# Autodesk Inventor assembly: ArcadeController
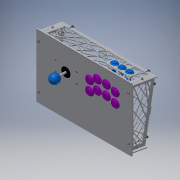
[picture p0: Inventor's stored thumbnail of the model, 180x180]
Saved by Autodesk Inventor 2019 (Build 230136000, 136)
## iProperties
Created: 2013-02-02
Part Number: ArcadeController
Document SubType Name: Assembly
Designer: xylzlyx
Author: xylzlyx
## Documents named in this file (14)
- D:\GitRepos\Pew-Pew-Stick\inventor\assemblies\ArcadeController.iam
- D:\GitRepos\Pew-Pew-Stick\inventor\parts\Panel_top.ipt
- D:\GitRepos\Pew-Pew-Stick\inventor\parts\Panel_bottom.ipt
- D:\GitRepos\Pew-Pew-Stick\inventor\parts\JLF-TP-8YT_body.ipt
- D:\GitRepos\Pew-Pew-Stick\inventor\parts\JLF-TP-8YT_ball.ipt
- D:\GitRepos\Pew-Pew-Stick\inventor\parts\JLF-TP-8YT_ring.ipt
- D:\GitRepos\Pew-Pew-Stick\inventor\parts\OBSF-30-B_button.ipt
- D:\GitRepos\Pew-Pew-Stick\inventor\parts\Panel_back.ipt
- D:\GitRepos\Pew-Pew-Stick\inventor\parts\Panel_front.ipt
- D:\GitRepos\Pew-Pew-Stick\inventor\parts\Panel_side.ipt
- D:\GitRepos\Pew-Pew-Stick\inventor\parts\OBSF-24_button.ipt
- C:\Users\mstine\Documents\Inventor\Content Center Files\R2019\en-US\ANSI B18.22.1\ANSI B18.22.1 - No. 6 - Type A.ipt
- C:\Users\mstine\Documents\Inventor\Content Center Files\R2019\en-US\ANSI B18.3(05)\ANSI B18.3 - 6-32 UNC - 0.5(31).ipt
- D:\GitRepos\Pew-Pew-Stick\inventor\assemblies\ArcadeController\Design Accelerator\Bolted Connection2.iam
## Components (53 placed, 13 different names)
1. TopPanel:1 — Flush:1, Flush:2, Insert:1, Insert:2, Insert:4, Insert:5, Insert:6, Insert:7, Insert:8, Insert:9, Insert:10, Insert:11, Insert:12, Mate:6, Mate:10, Insert:14, Insert:17, Insert:18, Insert:19, Mate:14, Mate:15
2. BottomPanel:1 — Flush:1, Flush:2, Mate:3, Flush:3, Flush:4, Flush:5, Flush:6, Flush:8, Flush:9, Mate:4, Mate:5, Flush:10, Flush:12, Flush:13, Mate:8, Flush:14, Mate:13, Insert:22, Insert:23, Insert:24, Insert:25, Insert:26, Insert:27, Insert:28, Insert:29
3. JLF-TP-8YT_body:1 — Insert:1, Insert:2, Insert:3, Mate:3
4. JoystickBall:1 — Insert:3
5. JoystickCover:1 — Insert:4
6. OBSF-30-B_button:1 — Insert:5
7. OBSF-30-B_button:2 — Insert:6
8. OBSF-30-B_button:3 — Insert:7
9. OBSF-30-B_button:4 — Insert:8
10. OBSF-30-B_button:5 — Insert:9
11. OBSF-30-B_button:6 — Insert:10
12. OBSF-30-B_button:7 — Insert:11
13. OBSF-30-B_button:8 — Insert:12
14. Panel_back:1 — Flush:3, Flush:4, Mate:5, Flush:10, Mate:11, Mate:12, Insert:15, Insert:16, Insert:45, Insert:46, Insert:47
15. Panel_front:1 — Flush:5, Flush:6, Flush:12, Mate:9, Flush:14, Mate:13, Insert:20, Insert:21
16. Panel_side:1 — Flush:8, Flush:9, Mate:4, Mate:6, Mate:12
17. Panel_side:2 — Flush:13, Mate:8, Mate:9, Mate:10, Mate:11
18. Hexagon Socket Head Cap Screw - Inch No. 6 - 32 UNC - 1/2:20 — Insert:13
19. Plain Washer (Inch) No. 6 - Type A:17 — Insert:13, Insert:14
20. Hexagon Socket Head Cap Screw - Inch No. 6 - 32 UNC - 1/2:21 — Insert:30
21. Plain Washer (Inch) No. 6 - Type A:18 — Insert:15, Insert:31
22. Hexagon Socket Head Cap Screw - Inch No. 6 - 32 UNC - 1/2:22 — Insert:31
23. Plain Washer (Inch) No. 6 - Type A:19 — Insert:16, Insert:30
24. Hexagon Socket Head Cap Screw - Inch No. 6 - 32 UNC - 1/2:23 — Insert:32
25. Plain Washer (Inch) No. 6 - Type A:20 — Insert:17, Insert:35
26. Hexagon Socket Head Cap Screw - Inch No. 6 - 32 UNC - 1/2:24 — Insert:33
27. Plain Washer (Inch) No. 6 - Type A:21 — Insert:19, Insert:32
28. Hexagon Socket Head Cap Screw - Inch No. 6 - 32 UNC - 1/2:25 — Insert:34
29. Plain Washer (Inch) No. 6 - Type A:22 — Insert:18, Insert:34
30. Plain Washer (Inch) No. 6 - Type A:23 — Insert:20, Insert:33
31. Plain Washer (Inch) No. 6 - Type A:24 — Insert:21, Insert:36
32. Plain Washer (Inch) No. 6 - Type A:25 — Insert:25, Insert:43
33. Plain Washer (Inch) No. 6 - Type A:26 — Insert:24, Insert:44
34. Plain Washer (Inch) No. 6 - Type A:27 — Insert:23, Insert:39
35. Plain Washer (Inch) No. 6 - Type A:28 — Insert:22, Insert:40
36. Plain Washer (Inch) No. 6 - Type A:29 — Insert:26, Insert:37
37. Plain Washer (Inch) No. 6 - Type A:30 — Insert:27, Insert:38
38. Plain Washer (Inch) No. 6 - Type A:31 — Insert:28, Insert:41
39. Plain Washer (Inch) No. 6 - Type A:32 — Insert:29, Insert:42
40. Hexagon Socket Head Cap Screw - Inch No. 6 - 32 UNC - 1/2:26 — Insert:40
41. Hexagon Socket Head Cap Screw - Inch No. 6 - 32 UNC - 1/2:27 — Insert:35
42. Hexagon Socket Head Cap Screw - Inch No. 6 - 32 UNC - 1/2:28 — Insert:36
43. Hexagon Socket Head Cap Screw - Inch No. 6 - 32 UNC - 1/2:29 — Insert:37
44. Hexagon Socket Head Cap Screw - Inch No. 6 - 32 UNC - 1/2:30 — Insert:39
45. Hexagon Socket Head Cap Screw - Inch No. 6 - 32 UNC - 1/2:31 — Insert:38
46. Hexagon Socket Head Cap Screw - Inch No. 6 - 32 UNC - 1/2:32 — Insert:42
47. Hexagon Socket Head Cap Screw - Inch No. 6 - 32 UNC - 1/2:33 — Insert:41
48. Hexagon Socket Head Cap Screw - Inch No. 6 - 32 UNC - 1/2:34 — Insert:43
49. Hexagon Socket Head Cap Screw - Inch No. 6 - 32 UNC - 1/2:35 — Insert:44
50. OBSF-24_button:1 — Insert:45
51. OBSF-24_button:2 — Insert:46
52. OBSF-24_button:3 — Insert:47
53. Bolted Connection:1 [sub-assembly] — Mate:14, Mate:15
## Relationships (71: Insert 47, Flush 12, Mate 12)
- Flush:1: TopPanel:1 ↔ BottomPanel:1
- Flush:2: TopPanel:1 ↔ BottomPanel:1
- Insert:1: TopPanel:1 ↔ JLF-TP-8YT_body:1
- Insert:2: TopPanel:1 ↔ JLF-TP-8YT_body:1
- Insert:3: JLF-TP-8YT_body:1 ↔ JoystickBall:1
- Insert:4: TopPanel:1 ↔ JoystickCover:1
- Insert:5: TopPanel:1 ↔ OBSF-30-B_button:1
- Insert:6: TopPanel:1 ↔ OBSF-30-B_button:2
- Insert:7: TopPanel:1 ↔ OBSF-30-B_button:3
- Insert:8: TopPanel:1 ↔ OBSF-30-B_button:4
- Insert:9: TopPanel:1 ↔ OBSF-30-B_button:5
- Insert:10: TopPanel:1 ↔ OBSF-30-B_button:6
- Insert:11: TopPanel:1 ↔ OBSF-30-B_button:7
- Insert:12: TopPanel:1 ↔ OBSF-30-B_button:8
- Mate:3 (44.45 mm): BottomPanel:1 ↔ JLF-TP-8YT_body:1
- Flush:3: BottomPanel:1 ↔ Panel_back:1
- Flush:4 (-12.7 mm): BottomPanel:1 ↔ Panel_back:1
- Flush:5: BottomPanel:1 ↔ Panel_front:1
- Flush:6 (-9.525 mm): BottomPanel:1 ↔ Panel_front:1
- Flush:8 (-9.525 mm): BottomPanel:1 ↔ Panel_side:1
- Flush:9 (9.525 mm): BottomPanel:1 ↔ Panel_side:1
- Mate:4: BottomPanel:1 ↔ Panel_side:1
- Mate:5: BottomPanel:1 ↔ Panel_back:1
- Flush:10: BottomPanel:1 ↔ Panel_back:1
- Mate:6: TopPanel:1 ↔ Panel_side:1
- Flush:12 (9.525 mm): BottomPanel:1 ↔ Panel_front:1
- Flush:13 (9.525 mm): BottomPanel:1 ↔ Panel_side:2
- Mate:8: BottomPanel:1 ↔ Panel_side:2
- Mate:9: Panel_front:1 ↔ Panel_side:2
- Mate:10: TopPanel:1 ↔ Panel_side:2
- Mate:11: Panel_back:1 ↔ Panel_side:2
- Mate:12: Panel_back:1 ↔ Panel_side:1
- Flush:14: BottomPanel:1 ↔ Panel_front:1
- Mate:13: BottomPanel:1 ↔ Panel_front:1
- Insert:13: Hexagon Socket Head Cap Screw - Inch No. 6 - 32 UNC - 1/2:20 ↔ Plain Washer (Inch) No. 6 - Type A:17
- Insert:14: TopPanel:1 ↔ Plain Washer (Inch) No. 6 - Type A:17
- Insert:15: Panel_back:1 ↔ Plain Washer (Inch) No. 6 - Type A:18
- Insert:16: Panel_back:1 ↔ Plain Washer (Inch) No. 6 - Type A:19
- Insert:17: TopPanel:1 ↔ Plain Washer (Inch) No. 6 - Type A:20
- Insert:18: TopPanel:1 ↔ Plain Washer (Inch) No. 6 - Type A:22
- Insert:19: TopPanel:1 ↔ Plain Washer (Inch) No. 6 - Type A:21
- Insert:20: Panel_front:1 ↔ Plain Washer (Inch) No. 6 - Type A:23
- Insert:21: Panel_front:1 ↔ Plain Washer (Inch) No. 6 - Type A:24
- Insert:22: BottomPanel:1 ↔ Plain Washer (Inch) No. 6 - Type A:28
- Insert:23: BottomPanel:1 ↔ Plain Washer (Inch) No. 6 - Type A:27
- Insert:24: BottomPanel:1 ↔ Plain Washer (Inch) No. 6 - Type A:26
- Insert:25: BottomPanel:1 ↔ Plain Washer (Inch) No. 6 - Type A:25
- Insert:26: BottomPanel:1 ↔ Plain Washer (Inch) No. 6 - Type A:29
- Insert:27: BottomPanel:1 ↔ Plain Washer (Inch) No. 6 - Type A:30
- Insert:28: BottomPanel:1 ↔ Plain Washer (Inch) No. 6 - Type A:31
- Insert:29: BottomPanel:1 ↔ Plain Washer (Inch) No. 6 - Type A:32
- Insert:30: Hexagon Socket Head Cap Screw - Inch No. 6 - 32 UNC - 1/2:21 ↔ Plain Washer (Inch) No. 6 - Type A:19
- Insert:31: Plain Washer (Inch) No. 6 - Type A:18 ↔ Hexagon Socket Head Cap Screw - Inch No. 6 - 32 UNC - 1/2:22
- Insert:32: Hexagon Socket Head Cap Screw - Inch No. 6 - 32 UNC - 1/2:23 ↔ Plain Washer (Inch) No. 6 - Type A:21
- Insert:33: Hexagon Socket Head Cap Screw - Inch No. 6 - 32 UNC - 1/2:24 ↔ Plain Washer (Inch) No. 6 - Type A:23
- Insert:34: Hexagon Socket Head Cap Screw - Inch No. 6 - 32 UNC - 1/2:25 ↔ Plain Washer (Inch) No. 6 - Type A:22
- Insert:35: Plain Washer (Inch) No. 6 - Type A:20 ↔ Hexagon Socket Head Cap Screw - Inch No. 6 - 32 UNC - 1/2:27
- Insert:36: Plain Washer (Inch) No. 6 - Type A:24 ↔ Hexagon Socket Head Cap Screw - Inch No. 6 - 32 UNC - 1/2:28
- Insert:37: Plain Washer (Inch) No. 6 - Type A:29 ↔ Hexagon Socket Head Cap Screw - Inch No. 6 - 32 UNC - 1/2:29
- Insert:38: Plain Washer (Inch) No. 6 - Type A:30 ↔ Hexagon Socket Head Cap Screw - Inch No. 6 - 32 UNC - 1/2:31
- Insert:39: Plain Washer (Inch) No. 6 - Type A:27 ↔ Hexagon Socket Head Cap Screw - Inch No. 6 - 32 UNC - 1/2:30
- Insert:40: Plain Washer (Inch) No. 6 - Type A:28 ↔ Hexagon Socket Head Cap Screw - Inch No. 6 - 32 UNC - 1/2:26
- Insert:41: Plain Washer (Inch) No. 6 - Type A:31 ↔ Hexagon Socket Head Cap Screw - Inch No. 6 - 32 UNC - 1/2:33
- Insert:42: Plain Washer (Inch) No. 6 - Type A:32 ↔ Hexagon Socket Head Cap Screw - Inch No. 6 - 32 UNC - 1/2:32
- Insert:43: Plain Washer (Inch) No. 6 - Type A:25 ↔ Hexagon Socket Head Cap Screw - Inch No. 6 - 32 UNC - 1/2:34
- Insert:44: Plain Washer (Inch) No. 6 - Type A:26 ↔ Hexagon Socket Head Cap Screw - Inch No. 6 - 32 UNC - 1/2:35
- Insert:45: Panel_back:1 ↔ OBSF-24_button:1
- Insert:46: Panel_back:1 ↔ OBSF-24_button:2
- Insert:47: Panel_back:1 ↔ OBSF-24_button:3
- Mate:14: TopPanel:1 ↔ Bolted Connection:1
- Mate:15: TopPanel:1 ↔ Bolted Connection:1
